# Autodesk Inventor assembly: back
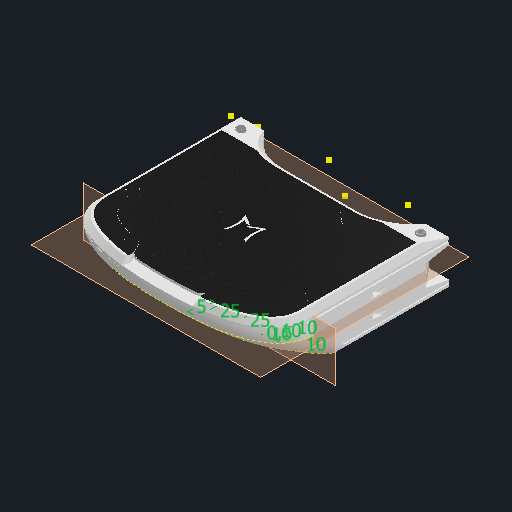
[picture p0: Inventor's stored thumbnail of the model, 512x512]
Saved by Autodesk Inventor 2025 (Build 290162000, 162)
## iProperties
Created: 2024-05-01
Part Number: back
Document SubType Name: Assembly
Designer: markm
Author: markm
## Documents named in this file (11)
- C:\Users\mark\OneDrive\Inventor\eventide\back\back.iam
- C:\Users\mark\OneDrive\Inventor\eventide\back\body.ipt
- C:\Users\mark\OneDrive\Inventor\eventide\back\cap.ipt
- C:\Users\mark\OneDrive\Inventor\Content Center Files\R2024\en-US\DIN 912\DIN 912 - M5 x 0,8 x 20 x 18.ipt
- C:\Users\mark\OneDrive\Inventor\eventide\back\battery\battery.iam
- C:\Users\mark\OneDrive\Inventor\eventide\back\lid.ipt
- C:\Users\mark\OneDrive\Inventor\eventide\back\socket\cap.ipt
- C:\Users\mark\OneDrive\Inventor\eventide\back\socket\MT60-F\MT60-F.ipt
- C:\Users\mark\OneDrive\Inventor\eventide\back\flank.ipt
- C:\Users\mark\OneDrive\Inventor\eventide\back\protection.ipt
- C:\Users\mark\OneDrive\Inventor\eventide\back\flank_MIR.ipt
## Components (21 placed, 9 different names)
1. body:1 — Flush:1, Mate:1, Mate:10, Mate:11, Mate:12, Mate:13, Mate:32, Mate:33, Mate:41, Mate:44, Flush:4, Mate:47, Mate:48, Mate:49, Mate:50, Mate:51
2. cap:1 — Flush:1, Mate:1, Mate:2, Mate:3, Mate:4, Mate:5, Mate:6, Mate:7, Mate:8, Mate:9, Flush:3, Mate:40, Mate:41, Mate:54, Mate:55, Mate:56
3. DIN 912 - replaced by DIN EN ISO 4762 M5 x 20:1 — Mate:10, Mate:13
4. DIN 912 - replaced by DIN EN ISO 4762 M5 x 20:2 — Mate:2, Mate:8
5. DIN 912 - replaced by DIN EN ISO 4762 M5 x 20:3 — Mate:3, Mate:7
6. DIN 912 - replaced by DIN EN ISO 4762 M5 x 20:4 — Mate:4, Mate:6
7. DIN 912 - replaced by DIN EN ISO 4762 M5 x 20:5 — Mate:5, Mate:9
8. DIN 912 - replaced by DIN EN ISO 4762 M5 x 20:8 — Mate:11, Mate:12
9. DIN 912 - replaced by DIN EN ISO 4762 M5 x 20:9
10. DIN 912 - replaced by DIN EN ISO 4762 M5 x 20:10
11. DIN 912 - replaced by DIN EN ISO 4762 M5 x 20:11
12. DIN 912 - replaced by DIN EN ISO 4762 M5 x 20:12
13. DIN 912 - replaced by DIN EN ISO 4762 M5 x 20:13
14. DIN 912 - replaced by DIN EN ISO 4762 M5 x 20:14
15. battery:1 [sub-assembly] — Mate:32, Mate:33, Mate:44
16. lid:1 — Flush:3, Mate:40
17. MT60-F:1 — Flush:4, Mate:47, Mate:48
18. cap:2 — Mate:49, Mate:50, Mate:51
19. flank:1 — Mate:54, Mate:55, Mate:56
20. protection:1
21. flank_MIR:1
## Relationships (29: Mate 26, Flush 3)
- Flush:1: body:1 ↔ cap:1
- Mate:1: body:1 ↔ cap:1
- Mate:2: cap:1 ↔ DIN 912 - replaced by DIN EN ISO 4762 M5 x 20:2
- Mate:3: cap:1 ↔ DIN 912 - replaced by DIN EN ISO 4762 M5 x 20:3
- Mate:4: cap:1 ↔ DIN 912 - replaced by DIN EN ISO 4762 M5 x 20:4
- Mate:5: cap:1 ↔ DIN 912 - replaced by DIN EN ISO 4762 M5 x 20:5
- Mate:6: cap:1 ↔ DIN 912 - replaced by DIN EN ISO 4762 M5 x 20:4
- Mate:7: cap:1 ↔ DIN 912 - replaced by DIN EN ISO 4762 M5 x 20:3
- Mate:8: cap:1 ↔ DIN 912 - replaced by DIN EN ISO 4762 M5 x 20:2
- Mate:9: cap:1 ↔ DIN 912 - replaced by DIN EN ISO 4762 M5 x 20:5
- Mate:10: body:1 ↔ DIN 912 - replaced by DIN EN ISO 4762 M5 x 20:1
- Mate:11: body:1 ↔ DIN 912 - replaced by DIN EN ISO 4762 M5 x 20:8
- Mate:12: body:1 ↔ DIN 912 - replaced by DIN EN ISO 4762 M5 x 20:8
- Mate:13: body:1 ↔ DIN 912 - replaced by DIN EN ISO 4762 M5 x 20:1
- Mate:32: body:1 ↔ battery:1
- Mate:33: body:1 ↔ battery:1
- Flush:3: cap:1 ↔ lid:1
- Mate:40: cap:1 ↔ lid:1
- Mate:41: body:1 ↔ cap:1
- Mate:44: body:1 ↔ battery:1
- Flush:4 (-2.5 mm): body:1 ↔ MT60-F:1
- Mate:47: body:1 ↔ MT60-F:1
- Mate:48: body:1 ↔ MT60-F:1
- Mate:49: body:1 ↔ cap:2
- Mate:50: body:1 ↔ cap:2
- Mate:51: body:1 ↔ cap:2
- Mate:54: cap:1 ↔ flank:1
- Mate:55: cap:1 ↔ flank:1
- Mate:56 (1.75 mm): cap:1 ↔ flank:1
